# Autodesk Inventor assembly: Final
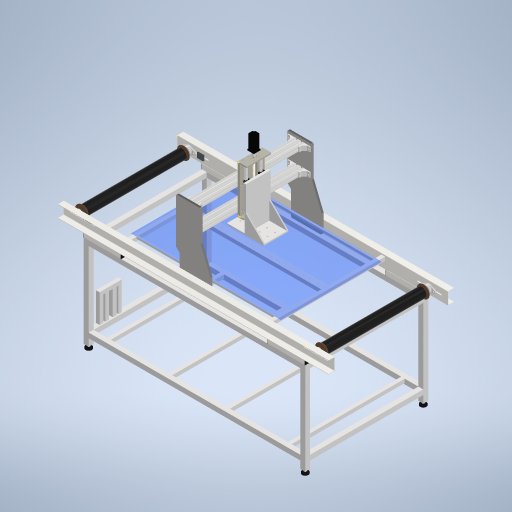
[picture p0: Inventor's stored thumbnail of the model, 512x512]
Saved by Autodesk Inventor 2023 (Build 270158000, 158)
## iProperties
Created: 2025-04-17
Part Number: Final
Document SubType Name: Assembly
Designer: huyqu
Author: huyqu
## Documents named in this file (3)
- E:\TAI LIEU\Final_Project\DONE\Final.iam
- E:\TAI LIEU\Final_Project\DONE\Bangtai\BangTai_Lap.iam
- E:\TAI LIEU\Final_Project\DONE\CoCauTrucZ\Co_Cau_Truc_Z.iam
## Components (2 placed, 2 different names)
1. BangTai_Lap:1 [sub-assembly] — Flush:1, Mate:1, Flush:2
2. Co_Cau_Truc_Z:1 [sub-assembly] — Flush:1, Mate:1, Flush:2
## Relationships (3: Flush 2, Mate 1)
- Flush:1: BangTai_Lap:1 ↔ Co_Cau_Truc_Z:1
- Mate:1: BangTai_Lap:1 ↔ Co_Cau_Truc_Z:1
- Flush:2 (940 mm): BangTai_Lap:1 ↔ Co_Cau_Truc_Z:1
